# Autodesk Inventor assembly: Glyf bot
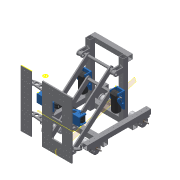
[picture p0: Inventor's stored thumbnail of the model, 180x180]
Saved by Autodesk Inventor 2018 (Build 220112000, 112)
## iProperties
Created: 2017-12-18
Part Number: Glyf bot
Document SubType Name: Assembly
Designer: dsayers
Author: dsayers
## Documents named in this file (21)
- C:\Fun Projects\FTC\Glyf bot.iam
- C:\Fun Projects\FTC\Drive Rail.ipt
- C:\Fun Projects\FTC\Drive Rail 1.ipt
- C:\Fun Projects\FTC\Motor.iam
- C:\Fun Projects\FTC\cube.ipt
- C:\Fun Projects\FTC\Drive Rail 1 upright.ipt
- C:\Fun Projects\FTC\Drive Rail 1 upright 2.ipt
- C:\Fun Projects\FTC\REV-41-1300.ipt
- C:\Fun Projects\FTC\momotr mount 2.ipt
- C:\Fun Projects\FTC\cross shaft.ipt
- C:\Fun Projects\FTC\cross beam.ipt
- C:\Fun Projects\FTC\Piv arm.ipt
- C:\Fun Projects\FTC\Top Piv.ipt
- C:\Fun Projects\FTC\cross shaft3.ipt
- C:\Fun Projects\FTC\Gripper Back.ipt
- C:\Fun Projects\FTC\grippy.ipt
- C:\Fun Projects\FTC\FTC Piv moount.ipt
- C:\Fun Projects\FTC\39172_txm-axle hub with set screw.ipt
- C:\Fun Projects\FTC\Clampy arm.ipt
- C:\Fun Projects\FTC\supporty.ipt
- C:\Fun Projects\FTC\supporty2.ipt
## Components (47 placed, 20 different names)
1. Drive Rail:1 — Flush:1, Flush:2, Mate:6, Flush:12, Mate:7, Mate:10, Flush:14, Symmetry:1, Flush:17, Mate:17, Flush:18, Mate:22, Angle:3
2. Drive Rail:2 — Flush:1, Flush:2, Mate:4, Mate:5, Mate:8, Flush:13, Symmetry:1, Mate:15, Flush:16, Mate:19, Mate:21
3. Drive Rail 1:1 — Mate:17, Mate:18, Flush:18
4. Drive Rail 1:2 — Mate:15, Flush:16, Flush:17, Mate:16, Mate:20, Flush:19, Flush:20, Mate:23
5. Motor:1 [sub-assembly] — Mate:4, Mate:5
6. Motor:2 [sub-assembly] — Mate:6, Flush:12, Mate:7, Mate:16
7. Motor:3 [sub-assembly] — Mate:10, Flush:14, Flush:15, Mate:18
8. Motor:4 [sub-assembly] — Mate:8, Flush:13, Flush:15, Mate:19, Mate:25
9. cube:1 — Mate:14, Mate:25, Mate:60, Flush:30, Flush:33, Angle:3
10. Drive Rail 1 upright:1 — Mate:22, Flush:20, Mate:23, Mate:24, Flush:21, Mate:28, Mate:52, Mate:114, Mate:117
11. Drive Rail 1 upright:2 — Mate:20, Mate:21, Flush:19, Flush:22, Mate:31, Angle:1, Mate:51, Mate:116, Mate:118
12. Drive Rail 1 upright 2:1 — Mate:24, Flush:21, Flush:22
13. REV-41-1300:1 — Mate:33, Mate:34, Flush:23
14. REV-41-1300:2 — Mate:35, Mate:36, Flush:23, Angle:1, Mate:37, Mate:38
15. momotr mount 2:1 — Mate:27, Mate:31, Mate:35, Mate:36, Flush:24, Mate:46, Mate:118
16. momotr mount 2:2 — Mate:27, Mate:28, Mate:33, Mate:34, Mate:41, Mate:114
17. cross shaft:1 — Mate:37, Mate:38, Flush:24, Mate:39, Mate:40
18. cross beam:1 — Mate:39, Mate:40, Mate:41, Flush:25, Flush:26
19. Piv arm:1 — Flush:25, Mate:47, Flush:27, Angle:2, Flush:40, Mate:106, Mate:107, Mate:109
20. Piv arm:2 — Flush:26, Mate:46, Mate:47, Flush:27, Mate:65, Mate:66, Flush:39, Mate:110, Mate:111, Mate:112, Mate:113
21. Top Piv:1 — Mate:51, Flush:28, Mate:116
22. Top Piv:2 — Mate:52, Mate:54, Mate:117
23. cross shaft3:1 — Mate:54, Flush:28, Mate:56, Mate:57
24. Piv arm:3 — Mate:56, Angle:2, Flush:40, Mate:97, Mate:98, Mate:100, Mate:101
25. Piv arm:4 — Mate:57, Mate:67, Flush:39, Mate:91, Mate:92, Mate:95
26. cube:2 — Mate:60, Flush:30, Mate:61, Flush:31, Flush:32, Flush:33
27. cube:3 — Mate:61, Flush:31, Flush:32, Mate:62
28. cube:4 — Mate:62
29. Gripper Back:1 — Mate:64, Mate:65, Mate:66, Mate:67, Mate:78, Mate:82, Flush:34, Flush:35, Flush:37, Mate:90, Mate:93, Mate:96, Mate:99, Mate:102, Mate:103, Mate:104, Mate:105, Mate:115, Mate:129, Mate:130, Mate:131, Mate:132, Mate:133, Mate:134
30. momotr mount 2:6 — Mate:75, Mate:76, Mate:77, Mate:78, Flush:35, Flush:36, Mate:115
31. REV-41-1300:5 — Mate:75, Mate:76, Mate:77
32. momotr mount 2:7 — Mate:82, Flush:34, Flush:36, Mate:119, Mate:120, Mate:126, Mate:128
33. REV-41-1300:6
34. grippy:1 — Flush:37, Mate:121, Mate:125, Mate:127, Mate:135
35. FTC Piv moount:1 — Mate:93, Mate:94, Mate:95
36. FTC Piv moount:2 — Mate:96, Mate:97, Mate:98
37. FTC Piv moount:3 — Mate:90, Mate:91, Mate:92, Mate:94
38. FTC Piv moount:4 — Mate:99, Mate:100, Mate:101
39. FTC Piv moount:5 — Mate:102, Mate:108, Mate:109
40. FTC Piv moount:6 — Mate:103, Mate:110, Mate:111
41. FTC Piv moount:7 — Mate:105, Mate:112, Mate:113
42. FTC Piv moount:8 — Mate:104, Mate:106, Mate:107, Mate:108
43. 39172_txm-axle hub with set screw:1 — Mate:119, Mate:120, Mate:121, Mate:123, Mate:124
44. Clampy arm:1 — Mate:126, Mate:127, Mate:128
45. Clampy arm:2 — Mate:123, Mate:124, Mate:125, Mate:135
46. supporty:1 — Mate:129, Mate:130, Mate:131
47. supporty2:1 — Mate:132, Mate:133, Mate:134
## Relationships (132: Mate 98, Flush 30, Angle 3, Symmetry 1)
- Flush:1: Drive Rail:1 ↔ Drive Rail:2
- Flush:2: Drive Rail:1 ↔ Drive Rail:2
- Mate:4: Drive Rail:2 ↔ Motor:1
- Mate:5: Drive Rail:2 ↔ Motor:1
- Mate:6: Drive Rail:1 ↔ Motor:2
- Flush:12: Drive Rail:1 ↔ Motor:2
- Mate:7: Drive Rail:1 ↔ Motor:2
- Mate:8: Drive Rail:2 ↔ Motor:4
- Flush:13: Drive Rail:2 ↔ Motor:4
- Mate:10: Drive Rail:1 ↔ Motor:3
- Flush:14: Drive Rail:1 ↔ Motor:3
- Flush:15: Motor:3 ↔ Motor:4
- Symmetry:1: Drive Rail:1 ↔ Drive Rail:2
- Mate:14 (-76.2 mm): cube:1
- Mate:15: Drive Rail:2 ↔ Drive Rail 1:2
- Flush:16: Drive Rail:2 ↔ Drive Rail 1:2
- Flush:17: Drive Rail:1 ↔ Drive Rail 1:2
- Mate:16: Drive Rail 1:2 ↔ Motor:2
- Mate:17: Drive Rail:1 ↔ Drive Rail 1:1
- Mate:18: Drive Rail 1:1 ↔ Motor:3
- Flush:18: Drive Rail:1 ↔ Drive Rail 1:1
- Mate:19: Drive Rail:2 ↔ Motor:4
- Mate:20: Drive Rail 1:2 ↔ Drive Rail 1 upright:2
- Mate:21: Drive Rail:2 ↔ Drive Rail 1 upright:2
- Flush:19: Drive Rail 1:2 ↔ Drive Rail 1 upright:2
- Mate:22: Drive Rail:1 ↔ Drive Rail 1 upright:1
- Flush:20: Drive Rail 1:2 ↔ Drive Rail 1 upright:1
- Mate:23: Drive Rail 1:2 ↔ Drive Rail 1 upright:1
- Mate:24: Drive Rail 1 upright:1 ↔ Drive Rail 1 upright 2:1
- Flush:21: Drive Rail 1 upright:1 ↔ Drive Rail 1 upright 2:1
- Flush:22: Drive Rail 1 upright:2 ↔ Drive Rail 1 upright 2:1
- Mate:25 (-50.8 mm): Motor:4 ↔ cube:1
- Mate:27: momotr mount 2:1 ↔ momotr mount 2:2
- Mate:28: Drive Rail 1 upright:1 ↔ momotr mount 2:2
- Mate:31: Drive Rail 1 upright:2 ↔ momotr mount 2:1
- Mate:33: REV-41-1300:1 ↔ momotr mount 2:2
- Mate:34: REV-41-1300:1 ↔ momotr mount 2:2
- Mate:35: REV-41-1300:2 ↔ momotr mount 2:1
- Mate:36: REV-41-1300:2 ↔ momotr mount 2:1
- Flush:23: REV-41-1300:1 ↔ REV-41-1300:2
- Angle:1 (90 deg): Drive Rail 1 upright:2 ↔ REV-41-1300:2
- Mate:37: REV-41-1300:2 ↔ cross shaft:1
- Mate:38: REV-41-1300:2 ↔ cross shaft:1
- Flush:24 (9.525 mm): momotr mount 2:1 ↔ cross shaft:1
- Mate:39: cross shaft:1 ↔ cross beam:1
- Mate:40: cross shaft:1 ↔ cross beam:1
- Mate:41 (3.175 mm): momotr mount 2:2 ↔ cross beam:1
- Flush:25: cross beam:1 ↔ Piv arm:1
- Flush:26: cross beam:1 ↔ Piv arm:2
- Mate:46: momotr mount 2:1 ↔ Piv arm:2
- Mate:47: Piv arm:1 ↔ Piv arm:2
- Flush:27: Piv arm:1 ↔ Piv arm:2
- Mate:51: Drive Rail 1 upright:2 ↔ Top Piv:1
- Mate:52: Drive Rail 1 upright:1 ↔ Top Piv:2
- Mate:54: Top Piv:2 ↔ cross shaft3:1
- Flush:28: Top Piv:1 ↔ cross shaft3:1
- [Mate]: Piv arm:3 ↔ Piv arm:4
- [Flush]: Piv arm:3 ↔ Piv arm:4
- Mate:56: cross shaft3:1 ↔ Piv arm:3
- Mate:57: cross shaft3:1 ↔ Piv arm:4
- Angle:2 (0 deg): Piv arm:1 ↔ Piv arm:3
- Mate:60: cube:1 ↔ cube:2
- Flush:30: cube:1 ↔ cube:2
- Mate:61: cube:2 ↔ cube:3
- Flush:31: cube:2 ↔ cube:3
- Flush:32: cube:2 ↔ cube:3
- Flush:33: cube:1 ↔ cube:2
- Angle:3 (0 deg): Drive Rail:1 ↔ cube:1
- Mate:62: cube:3 ↔ cube:4
- Mate:64 (-79.375 mm): Gripper Back:1
- Mate:65 (-38.1 mm): Piv arm:2 ↔ Gripper Back:1
- Mate:66 (19.05 mm): Piv arm:2 ↔ Gripper Back:1
- Mate:67 (19.05 mm): Piv arm:4 ↔ Gripper Back:1
- Mate:75: momotr mount 2:6 ↔ REV-41-1300:5
- Mate:76: momotr mount 2:6 ↔ REV-41-1300:5
- Mate:77: momotr mount 2:6 ↔ REV-41-1300:5
- Mate:78: Gripper Back:1 ↔ momotr mount 2:6
- [Mate]: momotr mount 2:7 ↔ REV-41-1300:6
- [Mate]: momotr mount 2:7 ↔ REV-41-1300:6
- [Mate]: momotr mount 2:7 ↔ REV-41-1300:6
- Mate:82: Gripper Back:1 ↔ momotr mount 2:7
- Flush:34 (-34.925 mm): Gripper Back:1 ↔ momotr mount 2:7
- Flush:35 (-34.925 mm): Gripper Back:1 ↔ momotr mount 2:6
- Flush:36: momotr mount 2:6 ↔ momotr mount 2:7
- Flush:37: Gripper Back:1 ↔ grippy:1
- Flush:39: Piv arm:2 ↔ Piv arm:4
- Flush:40: Piv arm:1 ↔ Piv arm:3
- Mate:90: Gripper Back:1 ↔ FTC Piv moount:3
- Mate:91: Piv arm:4 ↔ FTC Piv moount:3
- Mate:92: Piv arm:4 ↔ FTC Piv moount:3
- Mate:93: Gripper Back:1 ↔ FTC Piv moount:1
- Mate:94: FTC Piv moount:1 ↔ FTC Piv moount:3
- Mate:95: Piv arm:4 ↔ FTC Piv moount:1
- Mate:96: Gripper Back:1 ↔ FTC Piv moount:2
- Mate:97: Piv arm:3 ↔ FTC Piv moount:2
- Mate:98: Piv arm:3 ↔ FTC Piv moount:2
- Mate:99: Gripper Back:1 ↔ FTC Piv moount:4
- Mate:100: Piv arm:3 ↔ FTC Piv moount:4
- Mate:101: Piv arm:3 ↔ FTC Piv moount:4
- Mate:102: Gripper Back:1 ↔ FTC Piv moount:5
- Mate:103: Gripper Back:1 ↔ FTC Piv moount:6
- Mate:104: Gripper Back:1 ↔ FTC Piv moount:8
- Mate:105: Gripper Back:1 ↔ FTC Piv moount:7
- Mate:106: Piv arm:1 ↔ FTC Piv moount:8
- Mate:107: Piv arm:1 ↔ FTC Piv moount:8
- Mate:108: FTC Piv moount:5 ↔ FTC Piv moount:8
- Mate:109: Piv arm:1 ↔ FTC Piv moount:5
- Mate:110: Piv arm:2 ↔ FTC Piv moount:6
- Mate:111: Piv arm:2 ↔ FTC Piv moount:6
- Mate:112: Piv arm:2 ↔ FTC Piv moount:7
- Mate:113: Piv arm:2 ↔ FTC Piv moount:7
- Mate:114: Drive Rail 1 upright:1 ↔ momotr mount 2:2
- Mate:115: Gripper Back:1 ↔ momotr mount 2:6
- Mate:116: Drive Rail 1 upright:2 ↔ Top Piv:1
- Mate:117: Drive Rail 1 upright:1 ↔ Top Piv:2
- Mate:118: Drive Rail 1 upright:2 ↔ momotr mount 2:1
- Mate:119: momotr mount 2:7 ↔ 39172_txm-axle hub with set screw:1
- Mate:120: momotr mount 2:7 ↔ 39172_txm-axle hub with set screw:1
- Mate:121 (12.7 mm): grippy:1 ↔ 39172_txm-axle hub with set screw:1
- Mate:123: 39172_txm-axle hub with set screw:1 ↔ Clampy arm:2
- Mate:124: 39172_txm-axle hub with set screw:1 ↔ Clampy arm:2
- Mate:125: grippy:1 ↔ Clampy arm:2
- Mate:126: momotr mount 2:7 ↔ Clampy arm:1
- Mate:127: grippy:1 ↔ Clampy arm:1
- Mate:128 (88.9 mm): momotr mount 2:7 ↔ Clampy arm:1
- Mate:129: Gripper Back:1 ↔ supporty:1
- Mate:130: Gripper Back:1 ↔ supporty:1
- Mate:131: Gripper Back:1 ↔ supporty:1
- Mate:132: Gripper Back:1 ↔ supporty2:1
- Mate:133: Gripper Back:1 ↔ supporty2:1
- Mate:134: Gripper Back:1 ↔ supporty2:1
- Mate:135 (-9.525 mm): grippy:1 ↔ Clampy arm:2
## Named parameters: d94_d85 = 0 mm, d95_d84 = 0 mm, d133_d129 = 0 mm, d134_d130 = 0 mm, d135_d131 = 0 mm
